# Autodesk Inventor assembly: 110033226_iam_09_背流景觀
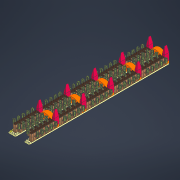
[picture p0: Inventor's stored thumbnail of the model, 180x180]
Saved by Autodesk Inventor 2022 (Build 260153000, 153)
## iProperties
Created: 2022-06-26
Part Number: 110033226_iam_09_背流景觀
Document SubType Name: Assembly
Designer: User
Author: User
## Documents named in this file (5)
- D:\D-disk\pomelo\大一\下學期\機械設計製圖\1100332260_LEGOproj_沒有公主城堡\110033226_iam_09_背流景觀.iam
- D:\D-disk\pomelo\大一\下學期\機械設計製圖\1100332260_LEGOproj_沒有公主城堡\110033226_ipt_39_背流基座.ipt
- D:\D-disk\pomelo\大一\下學期\機械設計製圖\1100332260_LEGOproj_沒有公主城堡\110033226_ipt_40_背流拱橋.ipt
- D:\D-disk\pomelo\大一\下學期\機械設計製圖\1100332260_LEGOproj_沒有公主城堡\110033226_ipt_38_小樹木.ipt
- D:\D-disk\pomelo\大一\下學期\機械設計製圖\1100332260_LEGOproj_沒有公主城堡\110033226_ipt_40_背流拱橋裝飾.ipt
## Components (166 placed, 4 different names)
1. 110033226_ipt_39_背流基座:1 — 貼合:1, 貼合:2, 貼合:3, 貼合:4, 貼合:5, 貼合:6, 貼合:7, 貼合:8, 對稱:1, 貼合:11, 貼合:12, 貼合:13, 貼合:14, 貼合:17, 貼合:19, 貼合:20
2. 110033226_ipt_40_背流拱橋裝飾:2 — 貼合:24, 貼合:25, 貼合:26
3. 110033226_ipt_40_背流拱橋:1 — 貼合:4, 貼合:5, 貼合:6, 貼合:9, 貼合:10, 貼合:15, 貼合:18, 貼合:22, 貼合:23, 貼合:24, 貼合:26
4. 110033226_ipt_40_背流拱橋裝飾:1 — 貼合:22, 貼合:23
5. 110033226_ipt_40_背流拱橋裝飾:3
6. 110033226_ipt_40_背流拱橋:2
7. 110033226_ipt_40_背流拱橋裝飾:4
8. 110033226_ipt_40_背流拱橋裝飾:5
9. 110033226_ipt_40_背流拱橋:3
10. 110033226_ipt_40_背流拱橋裝飾:6
11. 110033226_ipt_40_背流拱橋裝飾:7
12. 110033226_ipt_40_背流拱橋:4
13. 110033226_ipt_40_背流拱橋裝飾:8
14. 110033226_ipt_40_背流拱橋裝飾:9
15. 110033226_ipt_40_背流拱橋:5
16. 110033226_ipt_40_背流拱橋裝飾:10
17. 110033226_ipt_38_小樹木:2 — 貼合:12
18. 110033226_ipt_38_小樹木:1 — 對稱:1, 貼合:10, 貼合:11
19. 110033226_ipt_38_小樹木:3 — 貼合:7, 貼合:8, 貼合:9
20. 110033226_ipt_38_小樹木:6 — 貼合:19, 貼合:20, 貼合:21
21. 110033226_ipt_38_小樹木:5 — 貼合:16, 貼合:17, 貼合:18, 貼合:21, 貼合:25
22. 110033226_ipt_38_小樹木:4 — 貼合:13, 貼合:14, 貼合:15, 貼合:16
23. 110033226_ipt_38_小樹木:7
24. 110033226_ipt_38_小樹木:8
25. 110033226_ipt_38_小樹木:9
26. 110033226_ipt_38_小樹木:10
27. 110033226_ipt_38_小樹木:11
28. 110033226_ipt_38_小樹木:12
29. 110033226_ipt_38_小樹木:13
30. 110033226_ipt_38_小樹木:14
31. 110033226_ipt_38_小樹木:15
32. 110033226_ipt_38_小樹木:16
33. 110033226_ipt_38_小樹木:17
34. 110033226_ipt_38_小樹木:18
35. 110033226_ipt_38_小樹木:19
36. 110033226_ipt_38_小樹木:20
37. 110033226_ipt_38_小樹木:21
38. 110033226_ipt_38_小樹木:22
39. 110033226_ipt_38_小樹木:23
40. 110033226_ipt_38_小樹木:24
41. 110033226_ipt_38_小樹木:25
42. 110033226_ipt_38_小樹木:26
43. 110033226_ipt_38_小樹木:27
44. 110033226_ipt_38_小樹木:28
45. 110033226_ipt_38_小樹木:29
46. 110033226_ipt_38_小樹木:30
47. 110033226_ipt_38_小樹木:31
48. 110033226_ipt_38_小樹木:32
49. 110033226_ipt_38_小樹木:33
50. 110033226_ipt_38_小樹木:34
51. 110033226_ipt_38_小樹木:35
52. 110033226_ipt_38_小樹木:36
53. 110033226_ipt_38_小樹木:37
54. 110033226_ipt_38_小樹木:38
55. 110033226_ipt_38_小樹木:39
56. 110033226_ipt_38_小樹木:40
57. 110033226_ipt_38_小樹木:41
58. 110033226_ipt_38_小樹木:42
59. 110033226_ipt_38_小樹木:43
60. 110033226_ipt_38_小樹木:44
61. 110033226_ipt_38_小樹木:45
62. 110033226_ipt_38_小樹木:46
63. 110033226_ipt_38_小樹木:47
64. 110033226_ipt_38_小樹木:48
65. 110033226_ipt_38_小樹木:49
66. 110033226_ipt_38_小樹木:50
67. 110033226_ipt_38_小樹木:51
68. 110033226_ipt_38_小樹木:52
69. 110033226_ipt_38_小樹木:53
70. 110033226_ipt_38_小樹木:54
71. 110033226_ipt_38_小樹木:55
72. 110033226_ipt_38_小樹木:56
73. 110033226_ipt_38_小樹木:57
74. 110033226_ipt_38_小樹木:58
75. 110033226_ipt_38_小樹木:59
76. 110033226_ipt_38_小樹木:60
77. 110033226_ipt_38_小樹木:61
78. 110033226_ipt_38_小樹木:62
79. 110033226_ipt_38_小樹木:63
80. 110033226_ipt_38_小樹木:64
81. 110033226_ipt_38_小樹木:65
82. 110033226_ipt_38_小樹木:66
83. 110033226_ipt_38_小樹木:67
84. 110033226_ipt_38_小樹木:68
85. 110033226_ipt_38_小樹木:69
86. 110033226_ipt_38_小樹木:70
87. 110033226_ipt_38_小樹木:71
88. 110033226_ipt_38_小樹木:72
89. 110033226_ipt_38_小樹木:73
90. 110033226_ipt_38_小樹木:74
91. 110033226_ipt_38_小樹木:75
92. 110033226_ipt_38_小樹木:76
93. 110033226_ipt_38_小樹木:77
94. 110033226_ipt_38_小樹木:78
95. 110033226_ipt_38_小樹木:79
96. 110033226_ipt_38_小樹木:80
97. 110033226_ipt_38_小樹木:81
98. 110033226_ipt_38_小樹木:82
99. 110033226_ipt_38_小樹木:83
100. 110033226_ipt_38_小樹木:84
101. 110033226_ipt_38_小樹木:85
102. 110033226_ipt_38_小樹木:86
103. 110033226_ipt_38_小樹木:87
104. 110033226_ipt_38_小樹木:88
105. 110033226_ipt_38_小樹木:89
106. 110033226_ipt_38_小樹木:90
107. 110033226_ipt_38_小樹木:91
108. 110033226_ipt_38_小樹木:92
109. 110033226_ipt_38_小樹木:93
110. 110033226_ipt_38_小樹木:94
111. 110033226_ipt_38_小樹木:95
112. 110033226_ipt_38_小樹木:96
113. 110033226_ipt_38_小樹木:97
114. 110033226_ipt_38_小樹木:98
115. 110033226_ipt_38_小樹木:99
116. 110033226_ipt_38_小樹木:100
117. 110033226_ipt_38_小樹木:101
118. 110033226_ipt_38_小樹木:102
119. 110033226_ipt_38_小樹木:103
120. 110033226_ipt_38_小樹木:104
121. 110033226_ipt_38_小樹木:105
122. 110033226_ipt_38_小樹木:106
123. 110033226_ipt_38_小樹木:107
124. 110033226_ipt_38_小樹木:108
125. 110033226_ipt_38_小樹木:109
126. 110033226_ipt_38_小樹木:110
127. 110033226_ipt_38_小樹木:111
128. 110033226_ipt_38_小樹木:112
129. 110033226_ipt_38_小樹木:113
130. 110033226_ipt_38_小樹木:114
131. 110033226_ipt_38_小樹木:115
132. 110033226_ipt_38_小樹木:116
133. 110033226_ipt_38_小樹木:117
134. 110033226_ipt_38_小樹木:118
135. 110033226_ipt_38_小樹木:119
136. 110033226_ipt_38_小樹木:120
137. 110033226_ipt_38_小樹木:121
138. 110033226_ipt_38_小樹木:122
139. 110033226_ipt_38_小樹木:123
140. 110033226_ipt_38_小樹木:124
141. 110033226_ipt_38_小樹木:125
142. 110033226_ipt_38_小樹木:126
143. 110033226_ipt_38_小樹木:127
144. 110033226_ipt_38_小樹木:128
145. 110033226_ipt_38_小樹木:129
146. 110033226_ipt_38_小樹木:130
147. 110033226_ipt_38_小樹木:131
148. 110033226_ipt_38_小樹木:132
149. 110033226_ipt_38_小樹木:133
150. 110033226_ipt_38_小樹木:134
151. 110033226_ipt_38_小樹木:135
152. 110033226_ipt_38_小樹木:136
153. 110033226_ipt_38_小樹木:137
154. 110033226_ipt_38_小樹木:138
155. 110033226_ipt_38_小樹木:139
156. 110033226_ipt_38_小樹木:140
157. 110033226_ipt_38_小樹木:141
158. 110033226_ipt_38_小樹木:142
159. 110033226_ipt_38_小樹木:143
160. 110033226_ipt_38_小樹木:144
161. 110033226_ipt_38_小樹木:145
162. 110033226_ipt_38_小樹木:146
163. 110033226_ipt_38_小樹木:147
164. 110033226_ipt_38_小樹木:148
165. 110033226_ipt_38_小樹木:149
166. 110033226_ipt_38_小樹木:150
## Component patterns: (5 elements, first: 110033226_ipt_40_背流拱橋裝飾:2 + 110033226_ipt_40_背流拱橋:1 + 110033226_ipt_40_背流拱橋裝飾:1), (5 elements, first: 110033226_ipt_38_小樹木:2 + 110033226_ipt_38_小樹木:1 + 110033226_ipt_38_小樹木:3 + 110033226_ipt_38_小樹木:6 + 110033226_ipt_38_小樹木:5 + 110033226_ipt_38_小樹木:4), 元件陣列 1:2 (5 elements), 元件陣列 1:3 (5 elements), 元件陣列 1:4 (5 elements), 元件陣列 1:5 (5 elements)
## Relationships (27: Mate 26, Symmetry 1)
- 貼合:1 [Mate]: 110033226_ipt_39_背流基座:1
- 貼合:2 [Mate]: 110033226_ipt_39_背流基座:1
- 貼合:3 [Mate]: 110033226_ipt_39_背流基座:1
- 貼合:4 [Mate]: 110033226_ipt_39_背流基座:1 ↔ 110033226_ipt_40_背流拱橋:1
- 貼合:5 [Mate]: 110033226_ipt_39_背流基座:1 ↔ 110033226_ipt_40_背流拱橋:1
- 貼合:6 [Mate]: 110033226_ipt_39_背流基座:1 ↔ 110033226_ipt_40_背流拱橋:1
- 貼合:7 [Mate]: 110033226_ipt_39_背流基座:1 ↔ 110033226_ipt_38_小樹木:3
- 貼合:8 [Mate]: 110033226_ipt_39_背流基座:1 ↔ 110033226_ipt_38_小樹木:3
- 貼合:9 [Mate]: 110033226_ipt_40_背流拱橋:1 ↔ 110033226_ipt_38_小樹木:3
- 對稱:1 [Symmetry]: 110033226_ipt_39_背流基座:1 ↔ 110033226_ipt_38_小樹木:1
- 貼合:10 [Mate]: 110033226_ipt_40_背流拱橋:1 ↔ 110033226_ipt_38_小樹木:1
- 貼合:11 [Mate]: 110033226_ipt_39_背流基座:1 ↔ 110033226_ipt_38_小樹木:1
- 貼合:12 [Mate]: 110033226_ipt_39_背流基座:1 ↔ 110033226_ipt_38_小樹木:2
- 貼合:13 [Mate]: 110033226_ipt_39_背流基座:1 ↔ 110033226_ipt_38_小樹木:4
- 貼合:14 [Mate]: 110033226_ipt_39_背流基座:1 ↔ 110033226_ipt_38_小樹木:4
- 貼合:15 [Mate]: 110033226_ipt_40_背流拱橋:1 ↔ 110033226_ipt_38_小樹木:4
- 貼合:16 [Mate]: 110033226_ipt_38_小樹木:5 ↔ 110033226_ipt_38_小樹木:4
- 貼合:17 [Mate]: 110033226_ipt_39_背流基座:1 ↔ 110033226_ipt_38_小樹木:5
- 貼合:18 [Mate]: 110033226_ipt_40_背流拱橋:1 ↔ 110033226_ipt_38_小樹木:5
- 貼合:19 [Mate]: 110033226_ipt_39_背流基座:1 ↔ 110033226_ipt_38_小樹木:6
- 貼合:20 [Mate]: 110033226_ipt_39_背流基座:1 ↔ 110033226_ipt_38_小樹木:6
- 貼合:21 [Mate]: 110033226_ipt_38_小樹木:6 ↔ 110033226_ipt_38_小樹木:5
- 貼合:22 [Mate]: 110033226_ipt_40_背流拱橋:1 ↔ 110033226_ipt_40_背流拱橋裝飾:1
- 貼合:23 [Mate]: 110033226_ipt_40_背流拱橋:1 ↔ 110033226_ipt_40_背流拱橋裝飾:1
- 貼合:24 [Mate]: 110033226_ipt_40_背流拱橋裝飾:2 ↔ 110033226_ipt_40_背流拱橋:1
- 貼合:25 [Mate]: 110033226_ipt_40_背流拱橋裝飾:2 ↔ 110033226_ipt_38_小樹木:5
- 貼合:26 [Mate]: 110033226_ipt_40_背流拱橋裝飾:2 ↔ 110033226_ipt_40_背流拱橋:1
